# Autodesk Inventor assembly: Wheel Insert Test Fit
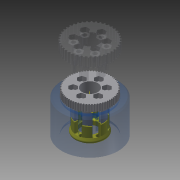
[picture p0: Inventor's stored thumbnail of the model, 180x180]
Saved by Autodesk Inventor 2015 (Build 190159000, 159)
## iProperties
Created: 2014-05-22
Part Number: Wheel Insert Test Fit
Document SubType Name: Assembly
Designer: dliu
Author: dliu
## Documents named in this file (5)
- C:\Users\dliu\Dropbox\dbhome\electric-longboard\dliu\Wheel Insert V3\Wheel Insert Test Fit V3.iam
- C:\Users\dliu\Dropbox\dbhome\electric-longboard\dliu\Board\Wheel Blank Pro 83mm.ipt
- C:\Users\dliu\Dropbox\dbhome\electric-longboard\dliu\Wheel Insert\Wheel Insert Retainer.ipt
- C:\Users\dliu\Dropbox\dbhome\electric-longboard\dliu\Wheel Insert\Wheel Insert Inner.ipt
- C:\Users\dliu\Dropbox\dbhome\electric-longboard\dliu\Wheel Insert V3\Wheel Insert Inner V3.ipt
## Components (4 placed, 4 different names)
1. Wheel Blank Pro 83mm:1
2. Wheel Insert Retainer:1 — Mate:1, Mate:2, Mate:7
3. Wheel Insert Inner:1 — Mate:4
4. Wheel Insert Inner V3:1 — Mate:6, Mate:7
## Relationships (5: Mate 5)
- Mate:1: Wheel Insert Retainer:1
- Mate:2: Wheel Insert Retainer:1
- Mate:4: Wheel Insert Inner:1
- Mate:6: Wheel Insert Inner V3:1
- Mate:7: Wheel Insert Retainer:1 ↔ Wheel Insert Inner V3:1
